# Autodesk Inventor assembly: DCMotorAssembly
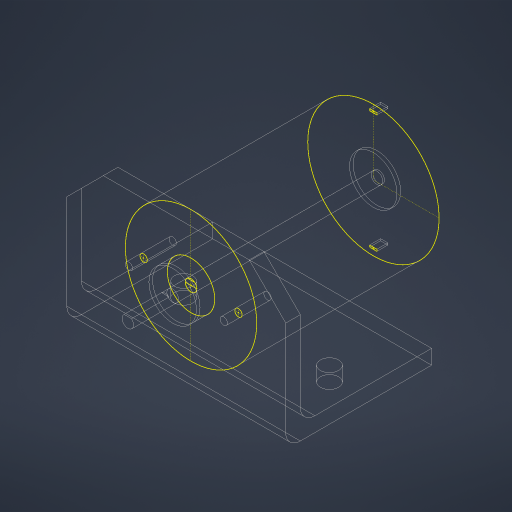
[picture p0: Inventor's stored thumbnail of the model, 512x512]
Saved by Autodesk Inventor 2023 (Build 270158000, 158)
## iProperties
Created: 2022-06-20
Part Number: DCMotorAssembly
Document SubType Name: Assembly
Designer: Levi
Mass: 184.131 g
Surface Area: 190.461 cm^2
Volume: 68.8672 cm^3
Density: 2.67371 g/cm^3
Author: Levi
## Documents named in this file (3)
- C:\Users\nleve\OneDrive\Desktop\szakdoga\modells\DCMotorAssembly.iam
- C:\Users\nleve\OneDrive\Desktop\szakdoga\modells\DCMotorPart.ipt
- C:\Users\nleve\OneDrive\Desktop\szakdoga\modells\MotorHolder-01.ipt
## Components (2 placed, 2 different names)
1. DCMotorPart:1 — Insert:1
2. MotorHolder-01:1 — Insert:1
## Relationships (1: Insert 1)
- Insert:1: DCMotorPart:1 ↔ MotorHolder-01:1
